# Autodesk Inventor assembly: Ring Drive
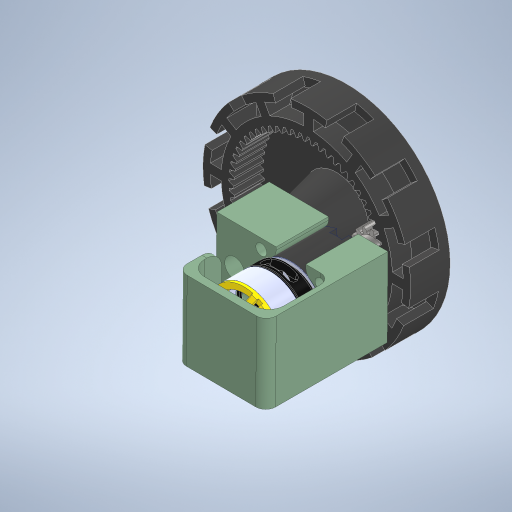
[picture p0: Inventor's stored thumbnail of the model, 512x512]
Saved by Autodesk Inventor 2023.2 (Build 272271000, 271)
## iProperties
Created: 2023-02-28
Part Number: Ring Drive
Document SubType Name: Assembly
Designer: Nathan Cai
Mass: 37.5513 g
Surface Area: 261.843 cm^2
Volume: 96.1759 cm^3
Density: 0.390443 g/cm^3
Author: Nathan Cai
## Documents named in this file (8)
- C:\Users\Nathan Cai\Documents\Inventor\Tests\Ring Drive\Ring Drive.iam
- C:\Users\Nathan Cai\Documents\Inventor\Tests\Ring Drive\RR Brushless\RR-Brushless-Planetary.iam
- C:\Users\Nathan Cai\Documents\Inventor\Tests\Ring Drive\4mmID 15T MOD0.8\2303-0004-0015 assembly.iam
- C:\Users\Nathan Cai\Documents\Inventor\Tests\Ring Drive\Temp - Gears.ipt
- C:\Users\Nathan Cai\Documents\Inventor\Tests\Ring Drive\Ring Drive\Design Accelerator\Spur Gears1.iam
- C:\Users\Nathan Cai\Documents\Inventor\Tests\Ring Drive\Ring Gear.ipt
- C:\Users\Nathan Cai\Documents\Inventor\Tests\Ring Drive\2938T1_High-Load Oil-Embedded Sleeve Bearing\2938T1_High-Load Oil-Embedded Sleeve Bearing.ipt
- C:\Users\Nathan Cai\Documents\Inventor\Asorted Parts\Pod.ipt
## Components (7 placed, 7 different names)
1. RR-Brushless-Planetary:1 [sub-assembly] — Mate:1, Mate:2, Mate:3, Mate:9, Flush:5
2. 2303-0004-0015 assembly:1 [sub-assembly] — Mate:1, Mate:2, Flush:2
3. Temp - Gears:1 — Mate:3, Mate:4, Mate:5, Mate:6, Flush:1, Mate:7
4. Spur Gears:1 [sub-assembly] — Mate:4, Mate:5, Mate:6, Flush:1, Flush:2
5. Spur Gear2:1 — Mate:7, Mate:8, Mate:11
6. 2938T1_High-Load Oil-Embedded Sleeve Bearing:1 — Mate:8, Mate:10
7. Pod:1 — Mate:9, Mate:10, Flush:5, Mate:11
## Relationships (14: Mate 11, Flush 3)
- Mate:1: RR-Brushless-Planetary:1 ↔ 2303-0004-0015 assembly:1
- Mate:2: RR-Brushless-Planetary:1 ↔ 2303-0004-0015 assembly:1
- Mate:3: RR-Brushless-Planetary:1 ↔ Temp - Gears:1
- Mate:4: Temp - Gears:1 ↔ Spur Gears:1
- Mate:5: Temp - Gears:1 ↔ Spur Gears:1
- Mate:6: Temp - Gears:1 ↔ Spur Gears:1
- Flush:1: Temp - Gears:1 ↔ Spur Gears:1
- Flush:2: 2303-0004-0015 assembly:1 ↔ Spur Gears:1
- Mate:7: Temp - Gears:1 ↔ Spur Gear2:1
- Mate:8: Spur Gear2:1 ↔ 2938T1_High-Load Oil-Embedded Sleeve Bearing:1
- Mate:9: RR-Brushless-Planetary:1 ↔ Pod:1
- Mate:10: 2938T1_High-Load Oil-Embedded Sleeve Bearing:1 ↔ Pod:1
- Flush:5: RR-Brushless-Planetary:1 ↔ Pod:1
- Mate:11 (6.35 mm): Spur Gear2:1 ↔ Pod:1
